# Autodesk Inventor assembly: 000.000 - Robot
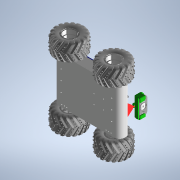
[picture p0: Inventor's stored thumbnail of the model, 180x180]
Saved by Autodesk Inventor 2022 (Build 260153000, 153)
## iProperties
Created: 2021-06-26
Part Number: 000.000 - Robot
Document SubType Name: Assembly
Designer: Петров Иван
Mass: 2460.21 g
Surface Area: 12880 cm^2
Volume: 1977.86 cm^3
Density: 1.24387 g/cm^3
Author: Петров Иван
## Documents named in this file (16)
- C:\git\4WDrobotFlask\000.000 - Robot.iam
- C:\git\4WDrobotFlask\000.001 - Bottom.ipt
- C:\git\4WDrobotFlask\боковая стенка.ipt
- C:\git\4WDrobotFlask\standart_components\01_Крепление_мотора.ipt
- C:\git\4WDrobotFlask\standart_components\JGA25-371_ASM\JGA25-371_ASM.iam
- C:\git\4WDrobotFlask\standart_components\WheelSmall\Wheel1.iam
- C:\git\4WDrobotFlask\000.002 - bamper.ipt
- C:\git\4WDrobotFlask\L298N Driver DC Motor, Stepper Motor.ipt
- C:\git\4WDrobotFlask\rpi3-bottom.ipt
- C:\git\4WDrobotFlask\battery_case.ipt
- C:\git\4WDrobotFlask\battery_case_top.ipt
- C:\git\4WDrobotFlask\rpi2-top_netfabb.ipt
- C:\git\4WDrobotFlask\C525.ipt
- C:\git\4WDrobotFlask\camera_holder.ipt
- C:\git\4WDrobotFlask\cam_hold_logitech.ipt
- C:\git\viki_mchs_robot\000.000 - Robot.iam
## Components (25 placed, 14 different names)
1. 000.001 - Bottom:1 — Совмещение:1, Заподлицо:2, Совмещение:2, Заподлицо:4, Заподлицо:6, Совмещение:3, Совмещение:4, Заподлицо:7, Заподлицо:9, Заподлицо:10, Заподлицо:11, Заподлицо:12, Заподлицо:13, Совмещение:25, Совмещение:26, Заподлицо:14, Совмещение:27, Совмещение:28, Заподлицо:15, Совмещение:35, Заподлицо:16
2. боковая стенка:1 — Заподлицо:9, Совмещение:32, Совмещение:33, Совмещение:34, Совмещение:36
3. 01_Крепление_мотора:1 — Совмещение:1, Заподлицо:2, Совмещение:5, Совмещение:6, Совмещение:7, Заподлицо:11, Совмещение:29
4. 01_Крепление_мотора:2 — Совмещение:2, Заподлицо:4, Совмещение:11, Совмещение:12, Совмещение:13, Заподлицо:10
5. 01_Крепление_мотора:3 — Заподлицо:6, Совмещение:3, Совмещение:8, Совмещение:9, Совмещение:10, Заподлицо:13
6. 01_Крепление_мотора:4 — Совмещение:4, Заподлицо:7, Совмещение:14, Совмещение:15, Совмещение:16, Заподлицо:12, Совмещение:32
7. JGA25-371_ASM:1 [sub-assembly] — Совмещение:5, Совмещение:6, Совмещение:7, Совмещение:21, Совмещение:22, Совмещение:30
8. JGA25-371_ASM:2 [sub-assembly] — Совмещение:8, Совмещение:9, Совмещение:10, Совмещение:17, Совмещение:18, Совмещение:34
9. JGA25-371_ASM:3 [sub-assembly] — Совмещение:11, Совмещение:12, Совмещение:13, Совмещение:23, Совмещение:24, Совмещение:31
10. JGA25-371_ASM:4 [sub-assembly] — Совмещение:14, Совмещение:15, Совмещение:16, Совмещение:19, Совмещение:20, Совмещение:33
11. Wheel1:1 [sub-assembly] — Совмещение:17, Совмещение:18, Касательность:2
12. Wheel1:2 [sub-assembly] — Совмещение:19, Совмещение:20
13. Wheel1:3 [sub-assembly] — Совмещение:21, Совмещение:22
14. Wheel1:4 [sub-assembly] — Совмещение:23, Совмещение:24, Касательность:1
15. боковая стенка:2 — Совмещение:29, Совмещение:30, Совмещение:31, Заподлицо:17
16. 000.002 - bamper:1 — Совмещение:25, Совмещение:26, Заподлицо:14
17. 000.002 - bamper:2 — Совмещение:27, Совмещение:28, Заподлицо:15, Совмещение:37
18. L298N Driver DC Motor, Stepper Motor:1 — Совмещение:35, Совмещение:36, Заподлицо:16
19. rpi3-bottom:1 — Совмещение:37, Заподлицо:17, Заподлицо:18, Заподлицо:20, Совмещение:38, Заподлицо:21, Заподлицо:22
20. battery_case:1 — Заподлицо:18, Заподлицо:19
21. battery_case_top:1 — Заподлицо:19
22. rpi2-top_netfabb:1 — Заподлицо:20, Совмещение:38, Заподлицо:21
23. camera_holder:1 — Заподлицо:22, Заподлицо:23
24. cam_hold_logitech:1 — Заподлицо:23, Совмещение:39, Заподлицо:24
25. C525:1 — Совмещение:39, Заподлицо:24
## Relationships (61: Mate 39, Flush 20, Tangent 2)
- Совмещение:1 [Mate]: 000.001 - Bottom:1 ↔ 01_Крепление_мотора:1
- Заподлицо:2 [Flush] (5 mm): 000.001 - Bottom:1 ↔ 01_Крепление_мотора:1
- Совмещение:2 [Mate]: 000.001 - Bottom:1 ↔ 01_Крепление_мотора:2
- Заподлицо:4 [Flush] (5 mm): 000.001 - Bottom:1 ↔ 01_Крепление_мотора:2
- Заподлицо:6 [Flush] (5 mm): 000.001 - Bottom:1 ↔ 01_Крепление_мотора:3
- Совмещение:3 [Mate]: 000.001 - Bottom:1 ↔ 01_Крепление_мотора:3
- Совмещение:4 [Mate]: 000.001 - Bottom:1 ↔ 01_Крепление_мотора:4
- Заподлицо:7 [Flush] (5 mm): 000.001 - Bottom:1 ↔ 01_Крепление_мотора:4
- Совмещение:5 [Mate]: 01_Крепление_мотора:1 ↔ JGA25-371_ASM:1
- Совмещение:6 [Mate]: 01_Крепление_мотора:1 ↔ JGA25-371_ASM:1
- Совмещение:7 [Mate]: 01_Крепление_мотора:1 ↔ JGA25-371_ASM:1
- Совмещение:8 [Mate]: 01_Крепление_мотора:3 ↔ JGA25-371_ASM:2
- Совмещение:9 [Mate]: 01_Крепление_мотора:3 ↔ JGA25-371_ASM:2
- Совмещение:10 [Mate]: 01_Крепление_мотора:3 ↔ JGA25-371_ASM:2
- Совмещение:11 [Mate]: 01_Крепление_мотора:2 ↔ JGA25-371_ASM:3
- Совмещение:12 [Mate]: 01_Крепление_мотора:2 ↔ JGA25-371_ASM:3
- Совмещение:13 [Mate]: 01_Крепление_мотора:2 ↔ JGA25-371_ASM:3
- Совмещение:14 [Mate]: 01_Крепление_мотора:4 ↔ JGA25-371_ASM:4
- Совмещение:15 [Mate]: 01_Крепление_мотора:4 ↔ JGA25-371_ASM:4
- Совмещение:16 [Mate]: 01_Крепление_мотора:4 ↔ JGA25-371_ASM:4
- Совмещение:17 [Mate]: JGA25-371_ASM:2 ↔ Wheel1:1
- Совмещение:18 [Mate]: JGA25-371_ASM:2 ↔ Wheel1:1
- Совмещение:19 [Mate]: JGA25-371_ASM:4 ↔ Wheel1:2
- Совмещение:20 [Mate]: JGA25-371_ASM:4 ↔ Wheel1:2
- Совмещение:21 [Mate]: JGA25-371_ASM:1 ↔ Wheel1:3
- Совмещение:22 [Mate]: JGA25-371_ASM:1 ↔ Wheel1:3
- Совмещение:23 [Mate]: JGA25-371_ASM:3 ↔ Wheel1:4
- Совмещение:24 [Mate]: JGA25-371_ASM:3 ↔ Wheel1:4
- Заподлицо:9 [Flush]: 000.001 - Bottom:1 ↔ боковая стенка:1
- Заподлицо:10 [Flush] (3 mm): 000.001 - Bottom:1 ↔ 01_Крепление_мотора:2
- Заподлицо:11 [Flush] (3 mm): 000.001 - Bottom:1 ↔ 01_Крепление_мотора:1
- Заподлицо:12 [Flush] (3 mm): 000.001 - Bottom:1 ↔ 01_Крепление_мотора:4
- Заподлицо:13 [Flush] (3 mm): 000.001 - Bottom:1 ↔ 01_Крепление_мотора:3
- Совмещение:25 [Mate]: 000.001 - Bottom:1 ↔ 000.002 - bamper:1
- Совмещение:26 [Mate]: 000.001 - Bottom:1 ↔ 000.002 - bamper:1
- Заподлицо:14 [Flush]: 000.001 - Bottom:1 ↔ 000.002 - bamper:1
- Совмещение:27 [Mate]: 000.001 - Bottom:1 ↔ 000.002 - bamper:2
- Совмещение:28 [Mate]: 000.001 - Bottom:1 ↔ 000.002 - bamper:2
- Заподлицо:15 [Flush]: 000.001 - Bottom:1 ↔ 000.002 - bamper:2
- Совмещение:29 [Mate]: 01_Крепление_мотора:1 ↔ боковая стенка:2
- Совмещение:30 [Mate]: JGA25-371_ASM:1 ↔ боковая стенка:2
- Совмещение:31 [Mate]: JGA25-371_ASM:3 ↔ боковая стенка:2
- Совмещение:32 [Mate]: боковая стенка:1 ↔ 01_Крепление_мотора:4
- Совмещение:33 [Mate]: боковая стенка:1 ↔ JGA25-371_ASM:4
- Совмещение:34 [Mate]: боковая стенка:1 ↔ JGA25-371_ASM:2
- Касательность:1 [Tangent]: Wheel1:4
- Касательность:2 [Tangent]: Wheel1:1
- Совмещение:35 [Mate] (2 mm): 000.001 - Bottom:1 ↔ L298N Driver DC Motor, Stepper Motor:1
- Совмещение:36 [Mate] (67 mm): боковая стенка:1 ↔ L298N Driver DC Motor, Stepper Motor:1
- Заподлицо:16 [Flush] (40 mm): 000.001 - Bottom:1 ↔ L298N Driver DC Motor, Stepper Motor:1
- Совмещение:37 [Mate]: 000.002 - bamper:2 ↔ rpi3-bottom:1
- Заподлицо:17 [Flush]: боковая стенка:2 ↔ rpi3-bottom:1
- Заподлицо:18 [Flush]: rpi3-bottom:1 ↔ battery_case:1
- Заподлицо:19 [Flush]: battery_case:1 ↔ battery_case_top:1
- Заподлицо:20 [Flush]: rpi3-bottom:1 ↔ rpi2-top_netfabb:1
- Совмещение:38 [Mate]: rpi3-bottom:1 ↔ rpi2-top_netfabb:1
- Заподлицо:21 [Flush]: rpi3-bottom:1 ↔ rpi2-top_netfabb:1
- Заподлицо:22 [Flush]: rpi3-bottom:1 ↔ camera_holder:1
- Заподлицо:23 [Flush]: camera_holder:1 ↔ cam_hold_logitech:1
- Совмещение:39 [Mate]: cam_hold_logitech:1 ↔ C525:1
- Заподлицо:24 [Flush]: cam_hold_logitech:1 ↔ C525:1
